# Autodesk Inventor assembly: Shoulder
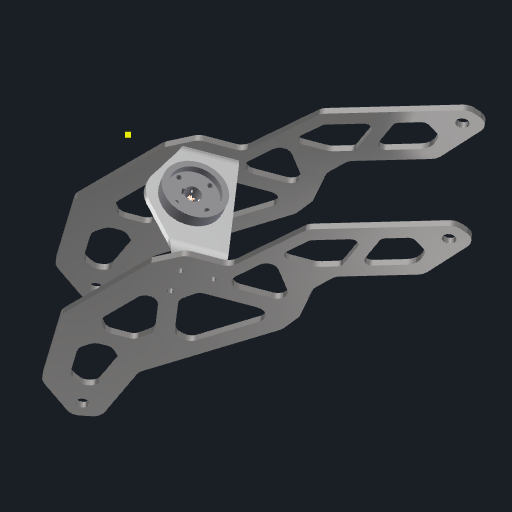
[picture p0: Inventor's stored thumbnail of the model, 512x512]
Saved by Autodesk Inventor 2023 (Build 270158000, 158)
## iProperties
Created: 2020-03-24
Part Number: Shoulder
Document SubType Name: Assembly
Designer: valer
Mass: 383.584 g
Surface Area: 442.479 cm^2
Volume: 56.5483 cm^3
Density: 6.7833 g/cm^3
Author: valer
## Documents named in this file (5)
- C:\Users\valer\Desktop\str1ker\cad\Shoulder.iam
- C:\Users\valer\Desktop\str1ker\cad\UpperArmBracket.ipt
- C:\Users\valer\Desktop\str1ker\cad\UpperArmBracketBase.ipt
- C:\Users\valer\Desktop\str1ker\cad\ShoulderBoundingBox.ipt
- C:\Users\valer\Desktop\str1ker\cad\BaseHub.ipt
## Components (5 placed, 4 different names)
1. UpperArmBracket:5 — Mate:386, Mate:387, Mate:392, Angle:1, Angle:3
2. UpperArmBracket:6 — Mate:384, Mate:385, Mate:391
3. UpperArmBracketBase:1 — Mate:384, Mate:385, Mate:386, Mate:387, Mate:391, Mate:392, Angle:2, Angle:4, Mate:394, Mate:395, Mate:396
4. ShoulderBoundingBox:1 — Mate:393, Angle:3, Angle:4
5. BaseHub:1 — Mate:394, Mate:395, Mate:396
## Relationships (14: Mate 10, Angle 4)
- Mate:384: UpperArmBracket:6 ↔ UpperArmBracketBase:1
- Mate:385: UpperArmBracket:6 ↔ UpperArmBracketBase:1
- Mate:386: UpperArmBracket:5 ↔ UpperArmBracketBase:1
- Mate:387: UpperArmBracket:5 ↔ UpperArmBracketBase:1
- Mate:391: UpperArmBracket:6 ↔ UpperArmBracketBase:1
- Mate:392: UpperArmBracket:5 ↔ UpperArmBracketBase:1
- Angle:1 (0 deg): UpperArmBracket:5
- Angle:2 (0 deg): UpperArmBracketBase:1
- Mate:393: ShoulderBoundingBox:1
- Angle:3 (0 deg): UpperArmBracket:5 ↔ ShoulderBoundingBox:1
- Angle:4 (0 deg): UpperArmBracketBase:1 ↔ ShoulderBoundingBox:1
- Mate:394: UpperArmBracketBase:1 ↔ BaseHub:1
- Mate:395: UpperArmBracketBase:1 ↔ BaseHub:1
- Mate:396: UpperArmBracketBase:1 ↔ BaseHub:1
